# Autodesk Inventor assembly: Tiger
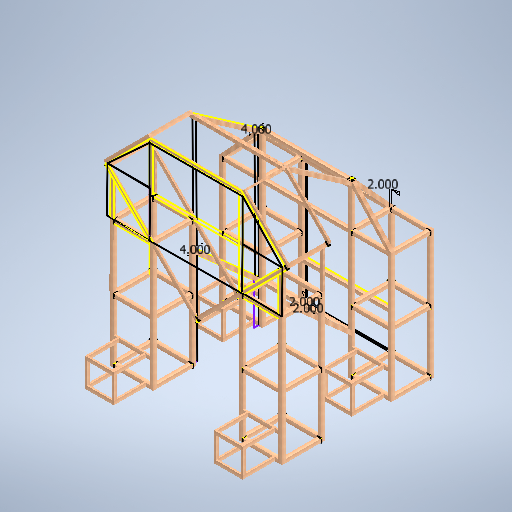
[picture p0: Inventor's stored thumbnail of the model, 512x512]
Saved by Autodesk Inventor 2025 (Build 290162000, 162)
## iProperties
Created: 2024-06-05
Part Number: Tiger
Document SubType Name: Assembly
Designer: Cupri
Mass: 180546 g
Surface Area: 136258 cm^2
Volume: 328266 cm^3
Density: 0.55 g/cm^3
Author: Cupri
## Documents named in this file (25)
- C:\Users\Cupri\OneDrive - University of South Carolina\Documents\Tiger\USCTigerBurn24\v2\Tiger.iam
- C:\Users\Cupri\OneDrive - University of South Carolina\Documents\Tiger\USCTigerBurn24\Standard Timber\4x4x72.ipt
- C:\Users\Cupri\OneDrive - University of South Carolina\Documents\Tiger\USCTigerBurn24\Standard Timber\4x4x40.ipt
- C:\Users\Cupri\OneDrive - University of South Carolina\Documents\Tiger\USCTigerBurn24\Standard Timber\2x4x36.ipt
- C:\Users\Cupri\OneDrive - University of South Carolina\Documents\Tiger\USCTigerBurn24\Standard Timber\2x4x40.ipt
- C:\Users\Cupri\OneDrive - University of South Carolina\Documents\Tiger\USCTigerBurn24\Standard Timber\2x4x24.ipt
- C:\Users\Cupri\OneDrive - University of South Carolina\Documents\Tiger\USCTigerBurn24\Standard Timber\2x4x28.ipt
- C:\Users\Cupri\OneDrive - University of South Carolina\Documents\Tiger\USCTigerBurn24\Standard Timber\2x4x72 (45 90).ipt
- C:\Users\Cupri\OneDrive - University of South Carolina\Documents\Tiger\USCTigerBurn24\Standard Timber\2x4x68 (45 90).ipt
- C:\Users\Cupri\OneDrive - University of South Carolina\Documents\Tiger\USCTigerBurn24\Standard Timber\2x4x42.343 (45 90).ipt
- C:\Users\Cupri\OneDrive - University of South Carolina\Documents\Tiger\USCTigerBurn24\Standard Timber\2x4x72 (30 90).ipt
- C:\Users\Cupri\OneDrive - University of South Carolina\Documents\Tiger\USCTigerBurn24\Standard Timber\2x4x44.ipt
- C:\Users\Cupri\OneDrive - University of South Carolina\Documents\Tiger\USCTigerBurn24\Standard Timber\4x4x104.303.ipt
- C:\Users\Cupri\OneDrive - University of South Carolina\Documents\Tiger\USCTigerBurn24\Standard Timber\4x4xidkanymore.ipt
- C:\Users\Cupri\OneDrive - University of South Carolina\Documents\Tiger\USCTigerBurn24\Standard Timber\4x4x48.ipt
- C:\Users\Cupri\OneDrive - University of South Carolina\Documents\Tiger\USCTigerBurn24\Standard Timber\4x4xigiveup.ipt
- C:\Users\Cupri\OneDrive - University of South Carolina\Documents\Tiger\USCTigerBurn24\Standard Timber\4x4x96.ipt
- C:\Users\Cupri\OneDrive - University of South Carolina\Documents\Tiger\USCTigerBurn24\Standard Timber\2x4x96.ipt
- C:\Users\Cupri\OneDrive - University of South Carolina\Documents\Tiger\USCTigerBurn24\Standard Timber\2x4xidk.ipt
- C:\Users\Cupri\OneDrive - University of South Carolina\Documents\Tiger\USCTigerBurn24\v2\Tiger\AIP\FEA\epzzwi8io.fins
- C:\Users\Cupri\OneDrive - University of South Carolina\Documents\Tiger\USCTigerBurn24\v2\Tiger\AIP\FEA\epzzwi8io.fsat
- C:\Users\Cupri\OneDrive - University of South Carolina\Documents\Tiger\USCTigerBurn24\v2\Tiger\AIP\FEA\epzzwi8io.ftes
- C:\Users\Cupri\OneDrive - University of South Carolina\Documents\Tiger\USCTigerBurn24\v2\Tiger\AIP\FEA\epzzwi8io.fwiz
- C:\Users\Cupri\OneDrive - University of South Carolina\Documents\Tiger\USCTigerBurn24\v2\Tiger\AIP\FEA\epzzwi8jk.fmsh
- C:\Users\Cupri\OneDrive - University of South Carolina\Documents\Tiger\USCTigerBurn24\v2\Tiger\AIP\FEA\epzzwi8jl.fres
## Components (160 placed, 18 different names)
1. 4x4x72:33 — Flush:163, Mate:149, Flush:164, Mate:182, Flush:229
2. 4x4x72:34 — Flush:161, Mate:148, Flush:162
3. 4x4x40:65
4. 4x4x40:66
5. 4x4x40:67
6. 4x4x40:68 — Flush:168
7. 4x4x40:69 — Flush:161
8. 4x4x40:70
9. 4x4x40:71
10. 4x4x40:72
11. 4x4x72:35 — Mate:150, Flush:165, Flush:166, Flush:224, Mate:181, Flush:227, Flush:228
12. 4x4x72:36 — Flush:158
13. 2x4x40:3
14. 2x4x36:9 — Mate:151
15. 2x4x36:10 — Flush:169, Flush:170
16. 2x4x36:11
17. 2x4x36:12
18. 2x4x24:5 — Flush:169
19. 2x4x24:6
20. 2x4x28:5 — Flush:170, Flush:200
21. 2x4x28:6 — Flush:167, Mate:151
22. 4x4x72:37 — Flush:163, Mate:149, Flush:164, Rigid:148, Flush:210, Mate:183, Flush:234
23. 4x4x72:38 — Mate:148, Flush:162
24. 4x4x40:77
25. 4x4x40:78
26. 4x4x40:79
27. 4x4x40:80 — Flush:231
28. 4x4x72:39 — Mate:150, Flush:165, Flush:166, Mate:172, Flush:215, Flush:216, Mate:184
29. 4x4x72:40 — Flush:158, Mate:173
30. 4x4x72:41
31. 4x4x72:42
32. 4x4x40:81
33. 4x4x40:82 — Flush:198
34. 4x4x40:83 — Flush:199
35. 4x4x40:84
36. 4x4x40:85
37. 4x4x40:86
38. 4x4x40:87
39. 4x4x40:88
40. 4x4x72:43
41. 4x4x72:44 — Flush:223
42. 2x4x40:4
43. 2x4x36:13
44. 2x4x36:14
45. 2x4x36:15
46. 2x4x36:16
47. 2x4x24:7
48. 2x4x24:8
49. 2x4x28:7 — Flush:200
50. 2x4x28:8
51. 4x4x72:45 — Flush:207
52. 4x4x72:46 — Flush:205, Rigid:147, Flush:211
53. 4x4x40:89 — Flush:206, Flush:212
54. 4x4x40:90 — Flush:208, Flush:209, Mate:176
55. 4x4x40:91 — Flush:205, Flush:207
56. 4x4x40:92 — Flush:206
57. 4x4x72:47 — Flush:208
58. 4x4x72:48 — Flush:209, Mate:171, Flush:213, Flush:214
59. 4x4x104.303:1 — Flush:221, Flush:222, Flush:224
60. 4x4x104.303:2 — Mate:179, Flush:220, Flush:221, Flush:222, Flush:223
61. 4x4xidkanymore:1 — Rigid:147, Flush:211, Flush:212
62. 4x4xidkanymore:2 — Rigid:148, Flush:210
63. 4x4x48:1 — Mate:172, Flush:215, Flush:216, Mate:174, Flush:217, Mate:180, Flush:225, Rigid:149, Flush:233, Mate:185, Flush:235, Flush:236
64. 4x4x48:2 — Mate:171, Flush:213, Flush:214, Mate:175, Flush:218, Rigid:150, Flush:226
65. 4x4xidkanymore:3 — Mate:173, Mate:174, Flush:217
66. 4x4xidkanymore:4 — Mate:175, Flush:218, Mate:176
67. 4x4xigiveup:1 — Mate:180, Flush:225, Rigid:149, Mate:186
68. 4x4xigiveup:2 — Rigid:150, Flush:226, Flush:237, Mate:187, Mate:188
69. 4x4x96:1 — Mate:183, Flush:231, Flush:232, Flush:234
70. 4x4x96:2 — Mate:184, Flush:232, Flush:233
71. 4x4x96:3 — Mate:181, Flush:227, Flush:228, Flush:230
72. 4x4x96:4 — Mate:182, Flush:229, Flush:230
73. 4x4x96:5 — Mate:185, Flush:235, Flush:236
74. 2x4x96:1 — Mate:186, Flush:237, Mate:187, Mate:188, Mate:191
75. 2x4xidk:1 — Mate:189, Mate:190, Mate:191, Flush:241
76. 2x4xidk:2 — Mate:192, Flush:240, Flush:241
77. 4x4x72:1 — Rigid:1, Rigid:3, Rigid:10, Rigid:11, Flush:39
78. 4x4x72:2 — Rigid:2, Rigid:4, Rigid:8
79. 4x4x40:1 — Rigid:1, Rigid:2
80. 4x4x40:2 — Rigid:3, Rigid:5, Flush:38, Mate:36
81. 4x4x40:3 — Rigid:6, Mate:5, Mate:6, Flush:4, Flush:5, Flush:19, Flush:20
82. 4x4x40:4 — Rigid:4, Rigid:7
83. 4x4x40:5 — Rigid:8
84. 4x4x40:6 — Rigid:9
85. 4x4x40:7 — Rigid:11
86. 4x4x40:8 — Rigid:10
87. 4x4x72:3 — Rigid:5, Rigid:6, Rigid:9, Mate:4, Flush:3, Mate:81
88. 4x4x72:4 — Rigid:7, Mate:7, Flush:21, Flush:22, Flush:159, Flush:160
89. 4x4x40:9
90. 4x4x40:10
91. 4x4x40:12 — Flush:168
92. 2x4x40:1 — Mate:4, Flush:3, Mate:5, Mate:8, Flush:6, Mate:9, Flush:7, Flush:17, Flush:18, Mate:81
93. 2x4x36:1 — Mate:6, Flush:4, Rigid:24, Flush:19, Flush:23
94. 2x4x36:2 — Mate:8, Flush:6, Flush:17, Mate:26, Mate:82
95. 2x4x36:3 — Mate:9, Flush:7, Mate:10, Rigid:26, Flush:18, Flush:21
96. 2x4x36:4 — Mate:7, Flush:5, Mate:10, Rigid:25, Rigid:27, Flush:20, Flush:22
97. 2x4x24:1 — Rigid:24, Mate:82
98. 2x4x24:2 — Rigid:25
99. 2x4x28:1 — Rigid:26, Mate:26
100. 2x4x28:2 — Rigid:27, Flush:23, Flush:167
101. 4x4x72:17 — Mate:62, Flush:65, Mate:63, Flush:91, Flush:92
102. 4x4x72:18 — Mate:64, Flush:66, Flush:90, Mate:76
103. 4x4x40:37 — Mate:75, Flush:89, Flush:90, Mate:76
104. 4x4x40:38 — Flush:85, Flush:86, Mate:74
105. 4x4x40:39 — Flush:92
106. 4x4x40:40 — Flush:91
107. 4x4x72:19 — Mate:38, Flush:41, Rigid:105, Mate:41, Flush:43, Flush:45, Flush:83, Flush:84, Flush:85
108. 4x4x72:20 — Mate:44, Flush:49, Flush:86, Flush:87, Mate:74, Mate:75, Flush:89, Flush:159, Flush:160
109. 4x4x72:21
110. 4x4x72:22 — Flush:39, Mate:77, Mate:179
111. 4x4x40:41
112. 4x4x40:42 — Flush:198
113. 4x4x40:43
114. 4x4x40:44 — Flush:38, Mate:36
115. 4x4x40:45
116. 4x4x40:46
117. 4x4x40:47
118. 4x4x40:48
119. 4x4x72:23 — Mate:78
120. 4x4x72:24
121. 4x4x40:49 — Flush:199
122. 4x4x40:50
123. 4x4x40:52
124. 2x4x40:2 — Mate:78, Mate:79, Mate:80
125. 2x4x36:5
126. 2x4x36:6 — Flush:50, Mate:47, Mate:80, Flush:95, Flush:96
127. 2x4x36:7 — Flush:93, Flush:94
128. 2x4x36:8
129. 2x4x24:3 — Mate:79
130. 2x4x24:4 — Flush:93, Flush:94
131. 2x4x28:3 — Flush:50, Mate:47, Flush:95, Flush:96
132. 2x4x28:4
133. 4x4x72:29 — Mate:57, Flush:57, Flush:58
134. 4x4x72:30 — Mate:58, Mate:60, Flush:60, Mate:77, Mate:178, Flush:220
135. 4x4x40:61
136. 4x4x40:62 — Flush:79, Flush:81, Mate:72
137. 4x4x40:63 — Flush:219, Mate:177, Mate:178
138. 4x4x40:64 — Mate:73
139. 4x4x72:31 — Mate:42, Mate:43, Flush:46, Flush:47, Flush:78, Flush:79, Mate:72, Mate:73
140. 4x4x72:32 — Mate:37, Flush:40, Rigid:104, Mate:39, Mate:40, Flush:42, Flush:80, Flush:81, Flush:82
141. 2x4x72 (45 90):1 — Mate:37, Flush:40, Rigid:104, Flush:80, Flush:88
142. 2x4x68 (45 90):1 — Mate:38, Flush:41, Rigid:105, Flush:44, Flush:83, Flush:88
143. 2x4x72 (45 90):2 — Mate:39, Mate:40, Flush:42, Flush:48, Mate:48, Flush:51, Mate:49, Flush:82
144. 2x4x72 (45 90):3 — Mate:41, Flush:43, Flush:44, Flush:45, Mate:45, Mate:50, Flush:52, Mate:51, Flush:84
145. 2x4x42.343 (45 90):1 — Mate:42, Mate:43, Flush:46, Flush:47, Flush:48, Flush:78
146. 2x4x42.343 (45 90):2 — Mate:44, Mate:45, Flush:49, Flush:87
147. 2x4x72 (30 90):1 — Mate:48, Flush:51, Mate:49, Flush:70, Flush:238, Mate:192, Flush:240
148. 2x4x72 (30 90):2 — Mate:50, Flush:52, Mate:51, Flush:71, Flush:72
149. 2x4x72 (45 90):4 — Mate:60, Flush:60, Mate:61, Flush:61, Flush:62
150. 2x4x68 (45 90):2 — Mate:61, Flush:61, Flush:62
151. 2x4x72 (45 90):5 — Flush:59, Mate:58, Mate:59, Mate:65, Flush:67, Flush:68, Flush:219, Mate:177
152. 2x4x72 (45 90):6 — Flush:63, Flush:64, Mate:62, Flush:65, Mate:63, Mate:68, Flush:73
153. 2x4x42.343 (45 90):3 — Mate:57, Flush:57, Flush:58, Flush:59, Mate:59
154. 2x4x42.343 (45 90):4 — Flush:63, Mate:64, Flush:66
155. 2x4x72 (30 90):3 — Mate:66, Flush:69, Flush:204, Mate:189
156. 2x4x72 (30 90):4 — Flush:64, Mate:67, Mate:69, Flush:239
157. 2x4x44:1 — Mate:67, Flush:71, Flush:72, Flush:239, Mate:190
158. 2x4x44:2 — Mate:65, Flush:67, Flush:68
159. 2x4x44:3 — Mate:66, Flush:69, Flush:70, Flush:204, Flush:238
160. 2x4x44:4 — Mate:68, Flush:73, Mate:69
## Relationships (372: Flush 176, Mate 114, WeldJoint 82)
- Rigid:1 [WeldJoint]: 4x4x72:1 ↔ 4x4x40:1
- Rigid:2 [WeldJoint]: 4x4x72:2 ↔ 4x4x40:1
- Rigid:3 [WeldJoint]: 4x4x72:1 ↔ 4x4x40:2
- Rigid:4 [WeldJoint]: 4x4x72:2 ↔ 4x4x40:4
- Rigid:5 [WeldJoint]: 4x4x40:2 ↔ 4x4x72:3
- Rigid:6 [WeldJoint]: 4x4x40:3 ↔ 4x4x72:3
- Rigid:7 [WeldJoint]: 4x4x40:4 ↔ 4x4x72:4
- Rigid:8 [WeldJoint]: 4x4x72:2 ↔ 4x4x40:5
- Rigid:9 [WeldJoint]: 4x4x40:6 ↔ 4x4x72:3
- Rigid:10 [WeldJoint]: 4x4x72:1 ↔ 4x4x40:8
- Rigid:11 [WeldJoint]: 4x4x72:1 ↔ 4x4x40:7
- Mate:4: 4x4x72:3 ↔ 2x4x40:1
- Flush:3: 4x4x72:3 ↔ 2x4x40:1
- Mate:5 (609.6 mm): 4x4x40:3 ↔ 2x4x40:1
- Mate:6 (101.6 mm): 4x4x40:3 ↔ 2x4x36:1
- Flush:4: 4x4x40:3 ↔ 2x4x36:1
- Mate:7 (101.6 mm): 4x4x72:4 ↔ 2x4x36:4
- Flush:5: 4x4x40:3 ↔ 2x4x36:4
- Mate:8 (101.6 mm): 2x4x40:1 ↔ 2x4x36:2
- Flush:6: 2x4x40:1 ↔ 2x4x36:2
- Mate:9: 2x4x40:1 ↔ 2x4x36:3
- Flush:7: 2x4x40:1 ↔ 2x4x36:3
- Mate:10: 2x4x36:3 ↔ 2x4x36:4
- Rigid:24 [WeldJoint]: 2x4x36:1 ↔ 2x4x24:1
- Rigid:25 [WeldJoint]: 2x4x36:4 ↔ 2x4x24:2
- Rigid:26 [WeldJoint]: 2x4x36:3 ↔ 2x4x28:1
- Rigid:27 [WeldJoint]: 2x4x36:4 ↔ 2x4x28:2
- [WeldJoint]: 4x4x72:18 ↔ 4x4x40:37
- [WeldJoint]: 4x4x40:38 ↔ 4x4x72:19
- [WeldJoint]: 4x4x72:17 ↔ 4x4x40:40
- [WeldJoint]: 4x4x72:17 ↔ 4x4x40:39
- Flush:17: 2x4x40:1 ↔ 2x4x36:2
- Flush:18: 2x4x40:1 ↔ 2x4x36:3
- Flush:19: 4x4x40:3 ↔ 2x4x36:1
- Flush:20: 4x4x40:3 ↔ 2x4x36:4
- Flush:21 (203.2 mm): 4x4x72:4 ↔ 2x4x36:3
- Flush:22 (203.2 mm): 4x4x72:4 ↔ 2x4x36:4
- Flush:23: 2x4x36:1 ↔ 2x4x28:2
- Mate:26: 2x4x36:2 ↔ 2x4x28:1
- [WeldJoint]: 4x4x72:21 ↔ 4x4x40:41
- [WeldJoint]: 4x4x72:22 ↔ 4x4x40:41
- [WeldJoint]: 4x4x72:21 ↔ 4x4x40:42
- [WeldJoint]: 4x4x72:22 ↔ 4x4x40:44
- [WeldJoint]: 4x4x40:42 ↔ 4x4x72:23
- [WeldJoint]: 4x4x40:43 ↔ 4x4x72:23
- [WeldJoint]: 4x4x40:44 ↔ 4x4x72:24
- [WeldJoint]: 4x4x72:22 ↔ 4x4x40:45
- [WeldJoint]: 4x4x40:46 ↔ 4x4x72:23
- [WeldJoint]: 4x4x72:21 ↔ 4x4x40:48
- [WeldJoint]: 4x4x72:21 ↔ 4x4x40:47
- [Mate]: 4x4x72:23 ↔ 2x4x40:2
- [Flush]: 4x4x72:23 ↔ 2x4x40:2
- [Mate] (609.6 mm): 4x4x40:43 ↔ 2x4x40:2
- [Mate] (101.6 mm): 4x4x40:43 ↔ 2x4x36:5
- [Flush]: 4x4x40:43 ↔ 2x4x36:5
- [Mate] (101.6 mm): 4x4x72:24 ↔ 2x4x36:8
- [Flush]: 4x4x40:43 ↔ 2x4x36:8
- [Mate]: 2x4x40:2 ↔ 2x4x36:7
- [Flush]: 2x4x40:2 ↔ 2x4x36:7
- [Mate]: 2x4x36:7 ↔ 2x4x36:8
- [WeldJoint]: 2x4x36:5 ↔ 2x4x24:3
- [WeldJoint]: 2x4x36:8 ↔ 2x4x24:4
- [WeldJoint]: 2x4x36:7 ↔ 2x4x28:3
- [WeldJoint]: 2x4x36:8 ↔ 2x4x28:4
- [WeldJoint]: 4x4x72:30 ↔ 4x4x40:61
- [WeldJoint]: 4x4x40:62 ↔ 4x4x72:31
- [WeldJoint]: 4x4x72:29 ↔ 4x4x40:64
- [WeldJoint]: 4x4x72:29 ↔ 4x4x40:63
- [Flush]: 2x4x40:2 ↔ 2x4x36:7
- [Flush]: 4x4x40:43 ↔ 2x4x36:5
- [Flush]: 4x4x40:43 ↔ 2x4x36:8
- [Flush] (203.2 mm): 4x4x72:24 ↔ 2x4x36:7
- [Flush] (203.2 mm): 4x4x72:24 ↔ 2x4x36:8
- [Flush]: 2x4x36:5 ↔ 2x4x28:4
- Flush:38: 4x4x40:2 ↔ 4x4x40:44
- Flush:39: 4x4x72:1 ↔ 4x4x72:22
- Mate:36 (2438.4 mm): 4x4x40:2 ↔ 4x4x40:44
- Mate:37: 4x4x72:32 ↔ 2x4x72 (45 90):1
- Flush:40: 4x4x72:32 ↔ 2x4x72 (45 90):1
- Rigid:104 [WeldJoint]: 4x4x72:32 ↔ 2x4x72 (45 90):1
- Mate:38: 4x4x72:19 ↔ 2x4x68 (45 90):1
- Flush:41: 4x4x72:19 ↔ 2x4x68 (45 90):1
- Rigid:105 [WeldJoint]: 4x4x72:19 ↔ 2x4x68 (45 90):1
- Mate:39: 4x4x72:32 ↔ 2x4x72 (45 90):2
- Mate:40: 4x4x72:32 ↔ 2x4x72 (45 90):2
- Flush:42: 4x4x72:32 ↔ 2x4x72 (45 90):2
- Mate:41: 4x4x72:19 ↔ 2x4x72 (45 90):3
- Flush:43: 4x4x72:19 ↔ 2x4x72 (45 90):3
- Flush:44: 2x4x68 (45 90):1 ↔ 2x4x72 (45 90):3
- Flush:45: 4x4x72:19 ↔ 2x4x72 (45 90):3
- Mate:42: 4x4x72:31 ↔ 2x4x42.343 (45 90):1
- Mate:43: 4x4x72:31 ↔ 2x4x42.343 (45 90):1
- Flush:46: 4x4x72:31 ↔ 2x4x42.343 (45 90):1
- Flush:47: 4x4x72:31 ↔ 2x4x42.343 (45 90):1
- Flush:48: 2x4x72 (45 90):2 ↔ 2x4x42.343 (45 90):1
- Mate:44: 4x4x72:20 ↔ 2x4x42.343 (45 90):2
- Mate:45: 2x4x72 (45 90):3 ↔ 2x4x42.343 (45 90):2
- Flush:49: 4x4x72:20 ↔ 2x4x42.343 (45 90):2
- Flush:50: 2x4x36:6 ↔ 2x4x28:3
- Mate:47: 2x4x36:6 ↔ 2x4x28:3
- Mate:48: 2x4x72 (45 90):2 ↔ 2x4x72 (30 90):1
- Flush:51: 2x4x72 (45 90):2 ↔ 2x4x72 (30 90):1
- Mate:49: 2x4x72 (45 90):2 ↔ 2x4x72 (30 90):1
- Mate:50: 2x4x72 (45 90):3 ↔ 2x4x72 (30 90):2
- Flush:52: 2x4x72 (45 90):3 ↔ 2x4x72 (30 90):2
- Mate:51: 2x4x72 (45 90):3 ↔ 2x4x72 (30 90):2
- [Flush]: 2x4x68 (45 90):2 ↔ 2x4x72 (45 90):6
- [Flush]: 2x4x72 (45 90):5 ↔ 2x4x42.343 (45 90):3
- [Mate]: 2x4x72 (45 90):6 ↔ 2x4x42.343 (45 90):4
- [Mate]: 2x4x72 (45 90):5 ↔ 2x4x72 (30 90):3
- [Flush]: 2x4x72 (45 90):5 ↔ 2x4x72 (30 90):3
- [Mate]: 2x4x72 (45 90):5 ↔ 2x4x72 (30 90):3
- [Mate]: 2x4x72 (45 90):6 ↔ 2x4x72 (30 90):4
- [Flush]: 2x4x72 (45 90):6 ↔ 2x4x72 (30 90):4
- [Mate]: 2x4x72 (45 90):6 ↔ 2x4x72 (30 90):4
- Mate:57: 4x4x72:29 ↔ 2x4x42.343 (45 90):3
- Flush:57: 4x4x72:29 ↔ 2x4x42.343 (45 90):3
- Flush:58: 4x4x72:29 ↔ 2x4x42.343 (45 90):3
- Flush:59: 2x4x72 (45 90):5 ↔ 2x4x42.343 (45 90):3
- Mate:58: 4x4x72:30 ↔ 2x4x72 (45 90):5
- Mate:59: 2x4x72 (45 90):5 ↔ 2x4x42.343 (45 90):3
- Mate:60: 4x4x72:30 ↔ 2x4x72 (45 90):4
- Flush:60: 4x4x72:30 ↔ 2x4x72 (45 90):4
- Mate:61: 2x4x72 (45 90):4 ↔ 2x4x68 (45 90):2
- Flush:61: 2x4x72 (45 90):4 ↔ 2x4x68 (45 90):2
- Flush:62: 2x4x72 (45 90):4 ↔ 2x4x68 (45 90):2
- Flush:63: 2x4x72 (45 90):6 ↔ 2x4x42.343 (45 90):4
- Flush:64: 2x4x72 (45 90):6 ↔ 2x4x72 (30 90):4
- Mate:62: 4x4x72:17 ↔ 2x4x72 (45 90):6
- Flush:65: 4x4x72:17 ↔ 2x4x72 (45 90):6
- Mate:63: 4x4x72:17 ↔ 2x4x72 (45 90):6
- Mate:64: 4x4x72:18 ↔ 2x4x42.343 (45 90):4
- Flush:66: 4x4x72:18 ↔ 2x4x42.343 (45 90):4
- Mate:65: 2x4x72 (45 90):5 ↔ 2x4x44:2
- Flush:67: 2x4x72 (45 90):5 ↔ 2x4x44:2
- Flush:68: 2x4x72 (45 90):5 ↔ 2x4x44:2
- Mate:66: 2x4x72 (30 90):3 ↔ 2x4x44:3
- Flush:69: 2x4x72 (30 90):3 ↔ 2x4x44:3
- Flush:70: 2x4x72 (30 90):1 ↔ 2x4x44:3
- Mate:67: 2x4x72 (30 90):4 ↔ 2x4x44:1
- Flush:71: 2x4x72 (30 90):2 ↔ 2x4x44:1
- Flush:72: 2x4x72 (30 90):2 ↔ 2x4x44:1
- Mate:68: 2x4x72 (45 90):6 ↔ 2x4x44:4
- Flush:73: 2x4x72 (45 90):6 ↔ 2x4x44:4
- Mate:69: 2x4x72 (30 90):4 ↔ 2x4x44:4
- Flush:78: 4x4x72:31 ↔ 2x4x42.343 (45 90):1
- Flush:79: 4x4x40:62 ↔ 4x4x72:31
- Flush:80: 4x4x72:32 ↔ 2x4x72 (45 90):1
- Flush:81: 4x4x40:62 ↔ 4x4x72:32
- Flush:82: 4x4x72:32 ↔ 2x4x72 (45 90):2
- Flush:83: 4x4x72:19 ↔ 2x4x68 (45 90):1
- Flush:84: 4x4x72:19 ↔ 2x4x72 (45 90):3
- Flush:85: 4x4x40:38 ↔ 4x4x72:19
- Flush:86: 4x4x40:38 ↔ 4x4x72:20
- Flush:87: 4x4x72:20 ↔ 2x4x42.343 (45 90):2
- Flush:88: 2x4x72 (45 90):1 ↔ 2x4x68 (45 90):1
- Mate:72: 4x4x40:62 ↔ 4x4x72:31
- Mate:73: 4x4x40:64 ↔ 4x4x72:31
- Mate:74: 4x4x40:38 ↔ 4x4x72:20
- Mate:75: 4x4x40:37 ↔ 4x4x72:20
- Flush:89: 4x4x40:37 ↔ 4x4x72:20
- Flush:90: 4x4x72:18 ↔ 4x4x40:37
- Mate:76: 4x4x72:18 ↔ 4x4x40:37
- Flush:91: 4x4x72:17 ↔ 4x4x40:40
- Flush:92: 4x4x72:17 ↔ 4x4x40:39
- Mate:77: 4x4x72:22 ↔ 4x4x72:30
- Mate:78: 4x4x72:23 ↔ 2x4x40:2
- Mate:79: 2x4x40:2 ↔ 2x4x24:3
- Flush:93: 2x4x36:7 ↔ 2x4x24:4
- Flush:94: 2x4x36:7 ↔ 2x4x24:4
- Mate:80: 2x4x40:2 ↔ 2x4x36:6
- Flush:95: 2x4x36:6 ↔ 2x4x28:3
- Flush:96: 2x4x36:6 ↔ 2x4x28:3
- Mate:81: 4x4x72:3 ↔ 2x4x40:1
- Mate:82: 2x4x36:2 ↔ 2x4x24:1
- [WeldJoint]: 4x4x72:33 ↔ 4x4x40:65
- [WeldJoint]: 4x4x72:34 ↔ 4x4x40:65
- [WeldJoint]: 4x4x72:33 ↔ 4x4x40:66
- [WeldJoint]: 4x4x72:34 ↔ 4x4x40:68
- [WeldJoint]: 4x4x40:66 ↔ 4x4x72:35
- [WeldJoint]: 4x4x40:67 ↔ 4x4x72:35
- [WeldJoint]: 4x4x40:68 ↔ 4x4x72:36
- [WeldJoint]: 4x4x72:34 ↔ 4x4x40:69
- [WeldJoint]: 4x4x40:70 ↔ 4x4x72:35
- [WeldJoint]: 4x4x72:33 ↔ 4x4x40:72
- [WeldJoint]: 4x4x72:33 ↔ 4x4x40:71
- [Mate]: 4x4x72:35 ↔ 2x4x40:3
- [Flush]: 4x4x72:35 ↔ 2x4x40:3
- [Mate] (609.6 mm): 4x4x40:67 ↔ 2x4x40:3
- [Mate] (101.6 mm): 4x4x40:67 ↔ 2x4x36:9
- [Flush]: 4x4x40:67 ↔ 2x4x36:9
- [Mate] (101.6 mm): 4x4x72:36 ↔ 2x4x36:12
- [Flush]: 4x4x40:67 ↔ 2x4x36:12
- [Mate] (101.6 mm): 2x4x40:3 ↔ 2x4x36:10
- [Flush]: 2x4x40:3 ↔ 2x4x36:10
- [Mate]: 2x4x40:3 ↔ 2x4x36:11
- [Flush]: 2x4x40:3 ↔ 2x4x36:11
- [Mate]: 2x4x36:11 ↔ 2x4x36:12
- [WeldJoint]: 2x4x36:9 ↔ 2x4x24:5
- [WeldJoint]: 2x4x36:12 ↔ 2x4x24:6
- [WeldJoint]: 2x4x36:11 ↔ 2x4x28:5
- [WeldJoint]: 2x4x36:12 ↔ 2x4x28:6
- [WeldJoint]: 4x4x72:38 ↔ 4x4x40:77
- [WeldJoint]: 4x4x40:78 ↔ 4x4x72:39
- [WeldJoint]: 4x4x72:37 ↔ 4x4x40:80
- [WeldJoint]: 4x4x72:37 ↔ 4x4x40:79
- [Flush]: 2x4x40:3 ↔ 2x4x36:10
- [Flush]: 2x4x40:3 ↔ 2x4x36:11
- [Flush]: 4x4x40:67 ↔ 2x4x36:9
- [Flush]: 4x4x40:67 ↔ 2x4x36:12
- [Flush] (203.2 mm): 4x4x72:36 ↔ 2x4x36:11
- [Flush] (203.2 mm): 4x4x72:36 ↔ 2x4x36:12
- [Flush]: 2x4x36:9 ↔ 2x4x28:6
- [Mate]: 2x4x36:10 ↔ 2x4x28:5
- [Flush]: 4x4x40:78 ↔ 4x4x72:39
- [Flush]: 4x4x40:78 ↔ 4x4x72:40
- [Mate]: 4x4x40:78 ↔ 4x4x72:40
- [Mate]: 4x4x40:77 ↔ 4x4x72:40
- [Flush]: 4x4x40:77 ↔ 4x4x72:40
- [Flush]: 4x4x72:38 ↔ 4x4x40:77
- [Mate]: 4x4x72:38 ↔ 4x4x40:77
- [Flush]: 4x4x72:37 ↔ 4x4x40:80
- [Flush]: 4x4x72:37 ↔ 4x4x40:79
- [Mate]: 4x4x72:35 ↔ 2x4x40:3
- [Mate]: 2x4x36:10 ↔ 2x4x24:5
- Flush:158: 4x4x72:36 ↔ 4x4x72:40
- Flush:159: 4x4x72:4 ↔ 4x4x72:20
- Flush:160: 4x4x72:4 ↔ 4x4x72:20
- Flush:161: 4x4x72:34 ↔ 4x4x40:69
- Mate:148: 4x4x72:34 ↔ 4x4x72:38
- Flush:162: 4x4x72:34 ↔ 4x4x72:38
- Flush:163: 4x4x72:33 ↔ 4x4x72:37
- Mate:149: 4x4x72:33 ↔ 4x4x72:37
- Flush:164: 4x4x72:33 ↔ 4x4x72:37
- Mate:150: 4x4x72:35 ↔ 4x4x72:39
- Flush:165: 4x4x72:35 ↔ 4x4x72:39
- Flush:166: 4x4x72:35 ↔ 4x4x72:39
- Flush:167: 2x4x28:6 ↔ 2x4x28:2
- Flush:168: 4x4x40:68 ↔ 4x4x40:12
- Mate:151: 2x4x36:9 ↔ 2x4x28:6
- Flush:169: 2x4x36:10 ↔ 2x4x24:5
- Flush:170: 2x4x36:10 ↔ 2x4x28:5
- [WeldJoint]: 4x4x72:41 ↔ 4x4x40:81
- [WeldJoint]: 4x4x72:42 ↔ 4x4x40:81
- [WeldJoint]: 4x4x72:41 ↔ 4x4x40:82
- [WeldJoint]: 4x4x72:42 ↔ 4x4x40:84
- [WeldJoint]: 4x4x40:82 ↔ 4x4x72:43
- [WeldJoint]: 4x4x40:83 ↔ 4x4x72:43
- [WeldJoint]: 4x4x40:84 ↔ 4x4x72:44
- [WeldJoint]: 4x4x72:42 ↔ 4x4x40:85
- [WeldJoint]: 4x4x40:86 ↔ 4x4x72:43
- [WeldJoint]: 4x4x72:41 ↔ 4x4x40:88
- [WeldJoint]: 4x4x72:41 ↔ 4x4x40:87
- [Mate]: 4x4x72:43 ↔ 2x4x40:4
- [Flush]: 4x4x72:43 ↔ 2x4x40:4
- [Mate] (609.6 mm): 4x4x40:83 ↔ 2x4x40:4
- [Mate] (101.6 mm): 4x4x40:83 ↔ 2x4x36:13
- [Flush]: 4x4x40:83 ↔ 2x4x36:13
- [Mate] (101.6 mm): 4x4x72:44 ↔ 2x4x36:16
- [Flush]: 4x4x40:83 ↔ 2x4x36:16
- [Mate] (101.6 mm): 2x4x40:4 ↔ 2x4x36:14
- [Flush]: 2x4x40:4 ↔ 2x4x36:14
- [Mate]: 2x4x40:4 ↔ 2x4x36:15
- [Flush]: 2x4x40:4 ↔ 2x4x36:15
- [Mate]: 2x4x36:15 ↔ 2x4x36:16
- [WeldJoint]: 2x4x36:13 ↔ 2x4x24:7
- [WeldJoint]: 2x4x36:16 ↔ 2x4x24:8
- [WeldJoint]: 2x4x36:15 ↔ 2x4x28:7
- [WeldJoint]: 2x4x36:16 ↔ 2x4x28:8
- [WeldJoint]: 4x4x72:46 ↔ 4x4x40:89
- [WeldJoint]: 4x4x40:90 ↔ 4x4x72:47
- [WeldJoint]: 4x4x72:45 ↔ 4x4x40:92
- [WeldJoint]: 4x4x72:45 ↔ 4x4x40:91
- [Flush]: 2x4x40:4 ↔ 2x4x36:14
- [Flush]: 2x4x40:4 ↔ 2x4x36:15
- [Flush]: 4x4x40:83 ↔ 2x4x36:13
- [Flush]: 4x4x40:83 ↔ 2x4x36:16
- [Flush] (203.2 mm): 4x4x72:44 ↔ 2x4x36:15
- [Flush] (203.2 mm): 4x4x72:44 ↔ 2x4x36:16
- [Flush]: 2x4x36:13 ↔ 2x4x28:8
- [Mate]: 2x4x36:14 ↔ 2x4x28:7
- [Flush]: 4x4x40:90 ↔ 4x4x72:47
- [Flush]: 4x4x40:90 ↔ 4x4x72:48
- [Mate]: 4x4x40:90 ↔ 4x4x72:48
- [Mate]: 4x4x40:89 ↔ 4x4x72:48
- [Flush]: 4x4x40:89 ↔ 4x4x72:48
- [Flush]: 4x4x72:46 ↔ 4x4x40:89
- [Mate]: 4x4x72:46 ↔ 4x4x40:89
- [Flush]: 4x4x72:45 ↔ 4x4x40:92
- [Flush]: 4x4x72:45 ↔ 4x4x40:91
- [Mate]: 4x4x72:43 ↔ 2x4x40:4
- [Mate]: 2x4x36:14 ↔ 2x4x24:7
- [Flush]: 4x4x72:44 ↔ 4x4x72:48
- [Flush]: 4x4x72:42 ↔ 4x4x40:85
- [Mate]: 4x4x72:42 ↔ 4x4x72:46
- [Flush]: 4x4x72:42 ↔ 4x4x72:46
- [Flush]: 4x4x72:41 ↔ 4x4x72:45
- [Mate]: 4x4x72:41 ↔ 4x4x72:45
- [Flush]: 4x4x72:41 ↔ 4x4x72:45
- [Mate]: 4x4x72:43 ↔ 4x4x72:47
- [Flush]: 4x4x72:43 ↔ 4x4x72:47
- [Flush]: 4x4x72:43 ↔ 4x4x72:47
- [Mate]: 2x4x36:13 ↔ 2x4x28:8
- [Flush]: 2x4x36:14 ↔ 2x4x24:7
- [Flush]: 2x4x36:14 ↔ 2x4x28:7
- Flush:198: 4x4x40:82 ↔ 4x4x40:42
- Flush:199: 4x4x40:83 ↔ 4x4x40:49
- Flush:200: 2x4x28:5 ↔ 2x4x28:7
- Flush:204: 2x4x72 (30 90):3 ↔ 2x4x44:3
- Flush:205: 4x4x72:46 ↔ 4x4x40:91
- Flush:206: 4x4x40:89 ↔ 4x4x40:92
- Flush:207: 4x4x72:45 ↔ 4x4x40:91
- Flush:208: 4x4x40:90 ↔ 4x4x72:47
- Flush:209: 4x4x40:90 ↔ 4x4x72:48
- Rigid:147 [WeldJoint]: 4x4x72:46 ↔ 4x4xidkanymore:1
- Rigid:148 [WeldJoint]: 4x4x72:37 ↔ 4x4xidkanymore:2
- Flush:210: 4x4x72:37 ↔ 4x4xidkanymore:2
- Flush:211: 4x4x72:46 ↔ 4x4xidkanymore:1
- Flush:212: 4x4x40:89 ↔ 4x4xidkanymore:1
- Mate:171: 4x4x72:48 ↔ 4x4x48:2
- Flush:213: 4x4x72:48 ↔ 4x4x48:2
- Flush:214: 4x4x72:48 ↔ 4x4x48:2
- Mate:172: 4x4x72:39 ↔ 4x4x48:1
- Flush:215: 4x4x72:39 ↔ 4x4x48:1
- Flush:216: 4x4x72:39 ↔ 4x4x48:1
- Mate:173: 4x4x72:40 ↔ 4x4xidkanymore:3
- Mate:174: 4x4x48:1 ↔ 4x4xidkanymore:3
- Flush:217: 4x4x48:1 ↔ 4x4xidkanymore:3
- Mate:175: 4x4x48:2 ↔ 4x4xidkanymore:4
- Flush:218: 4x4x48:2 ↔ 4x4xidkanymore:4
- Mate:176: 4x4x40:90 ↔ 4x4xidkanymore:4
- Flush:219: 4x4x40:63 ↔ 2x4x72 (45 90):5
- Mate:177: 4x4x40:63 ↔ 2x4x72 (45 90):5
- Mate:178: 4x4x72:30 ↔ 4x4x40:63
- Mate:179 (914.4 mm): 4x4x104.303:2 ↔ 4x4x72:22
- Flush:220: 4x4x104.303:2 ↔ 4x4x72:30
- Flush:221: 4x4x104.303:1 ↔ 4x4x104.303:2
- Flush:222: 4x4x104.303:1 ↔ 4x4x104.303:2
- Flush:223: 4x4x72:44 ↔ 4x4x104.303:2
- Flush:224: 4x4x72:35 ↔ 4x4x104.303:1
- Mate:180: 4x4x48:1 ↔ 4x4xigiveup:1
- Flush:225: 4x4x48:1 ↔ 4x4xigiveup:1
- Rigid:149 [WeldJoint]: 4x4x48:1 ↔ 4x4xigiveup:1
- Rigid:150 [WeldJoint]: 4x4x48:2 ↔ 4x4xigiveup:2
- Flush:226: 4x4x48:2 ↔ 4x4xigiveup:2
- Mate:181: 4x4x72:35 ↔ 4x4x96:3
- Flush:227: 4x4x72:35 ↔ 4x4x96:3
- Flush:228 (1053.8714 mm): 4x4x72:35 ↔ 4x4x96:3
- Mate:182: 4x4x72:33 ↔ 4x4x96:4
- Flush:229: 4x4x72:33 ↔ 4x4x96:4
- Flush:230: 4x4x96:3 ↔ 4x4x96:4
- Mate:183: 4x4x72:37 ↔ 4x4x96:1
- Mate:184: 4x4x72:39 ↔ 4x4x96:2
- Flush:231: 4x4x40:80 ↔ 4x4x96:1
- Flush:232: 4x4x96:1 ↔ 4x4x96:2
- Flush:233: 4x4x48:1 ↔ 4x4x96:2
- Flush:234: 4x4x72:37 ↔ 4x4x96:1
- Mate:185: 4x4x48:1 ↔ 4x4x96:5
- Flush:235: 4x4x48:1 ↔ 4x4x96:5
- Flush:236: 4x4x48:1 ↔ 4x4x96:5
- Mate:186: 4x4xigiveup:1 ↔ 2x4x96:1
- Flush:237: 4x4xigiveup:2 ↔ 2x4x96:1
- Mate:187: 4x4xigiveup:2 ↔ 2x4x96:1
- Mate:188: 4x4xigiveup:2 ↔ 2x4x96:1
- Flush:238: 2x4x72 (30 90):1 ↔ 2x4x44:3
- Flush:239: 2x4x72 (30 90):4 ↔ 2x4x44:1
- Mate:189: 2x4xidk:1 ↔ 2x4x72 (30 90):3
- Mate:190: 2x4xidk:1 ↔ 2x4x44:1
- Mate:191: 2x4x96:1 ↔ 2x4xidk:1
- Mate:192: 2x4xidk:2 ↔ 2x4x72 (30 90):1
- Flush:240: 2x4xidk:2 ↔ 2x4x72 (30 90):1
- Flush:241: 2x4xidk:1 ↔ 2x4xidk:2
## Named parameters: sa_0 = 22241.1, d136_d47_d36 = 0 mm, d137_d48_d37 = 0 mm, d138_d49_d38 = 0 mm, d139_d50_d39 = 0 mm, d154_d144 = 0 mm, d155_d145 = 0 mm, d156_d146 = 0 mm, d157_d147 = 203.2 mm, d158_d148 = 203.2 mm, d159_d149 = 0 mm, d168_d136_d47_d36 = 0 mm, d169_d137_d48_d37 = 0 mm, d170_d138_d49_d38 = 0 mm, d171_d139_d50_d39 = 0 mm, d173_d61 = 0 mm, d174_d62 = 0 mm, d175_d63 = 609.6 mm, d176_d68 = 101.6 mm, d177_d69 = 0 mm, d178_d70 = 101.6 mm, d179_d71 = 0 mm, d182_d74 = 0 mm, d183_d75 = 0 mm, d184_d76 = 0 mm, d185_d77 = 0 mm, d186_d78 = 0 mm, d187_d79 = 0 mm, d188_d80 = 0 mm, d190_d31 = 0 mm, d191_d32 = 0 mm, d192_d33 = 0 mm, d193_d34 = 0 mm, d194_d35 = 0 mm, d195_d36 = 0 mm, d196_d37 = 0 mm, d197_d38 = 0 mm, d198_d39 = 0 mm, d210_d29 = 0 mm, d211_d30 = 0 mm, d253_d234 = 0 mm, d254_d240 = 0 mm, d255_d242 = 0 mm, d256_d247 = 0 mm, d257_d248 = 0 mm, d258_d249 = 0 mm, d259_d250 = 0 mm, d260_d251 = 0 mm, d261_d252 = 0 mm, sa_1 = 980.999, d396_d137_d48_d37 = 0 mm, d397_d138_d49_d38 = 0 mm, d398_d139_d50_d39 = 0 mm, d399_d143 = 0 mm, d400_d144 = 0 mm, d401_d145 = 0 mm, d402_d146 = 0 mm, d403_d147 = 203.2 mm, d404_d148 = 203.2 mm, d405_d149 = 0 mm, d406_d150 = 0 mm, d407_d61 = 0 mm, d408_d62 = 0 mm, d409_d63 = 609.6 mm, d410_d68 = 101.6 mm, d411_d69 = 0 mm, d412_d70 = 101.6 mm, d413_d71 = 0 mm, d414_d72 = 101.6 mm, d415_d73 = 0 mm, d416_d74 = 0 mm, d417_d75 = 0 mm, d418_d76 = 0 mm, d419_d77 = 0 mm, d420_d78 = 0 mm, d421_d79 = 0 mm, d422_d80 = 0 mm, d423_d136_d47_d36 = 0 mm, d425_d31 = 0 mm, d426_d32 = 0 mm, d427_d33 = 0 mm, d428_d34 = 0 mm, d429_d35 = 0 mm, d430_d36 = 0 mm, d431_d37 = 0 mm, d432_d38 = 0 mm, d433_d39 = 0 mm, d434_d29 = 0 mm, d435_d30 = 0 mm, d436_d326 = 0 mm, d437_d327 = 0 mm, d438_d314 = 0 mm, d439_d315 = 0 mm, d440_d316 = 0 mm, d441_d317 = 0 mm, d442_d305 = 0 mm, d443_d306 = 0 mm, d444_d311 = 0 mm, d445_d312 = 0 mm, d446_d313 = 0 mm, d515_d433_d39 = 0 mm, d516_d434_d29 = 0 mm, d517_d435_d30 = 0 mm, d518_d436_d326 = 0 mm, d519_d437_d327 = 0 mm, d520_d438_d314 = 0 mm, d521_d439_d315 = 0 mm, d522_d440_d316 = 0 mm, d523_d441_d317 = 0 mm, d524_d442_d305 = 0 mm, d525_d443_d306 = 0 mm, d526_d444_d311 = 0 mm, d527_d445_d312 = 0 mm, d528_d446_d313 = 0 mm, d529_d396_d137_d48_d37 = 0 mm, d530_d397_d138_d49_d38 = 0 mm, d531_d398_d139_d50_d39 = 0 mm, d532_d399_d143 = 0 mm, d533_d400_d144 = 0 mm, d534_d401_d145 = 0 mm, d535_d402_d146 = 0 mm, d536_d403_d147 = 203.2 mm, d537_d404_d148 = 203.2 mm, d538_d405_d149 = 0 mm, d539_d406_d150 = 0 mm, d540_d407_d61 = 0 mm, d541_d408_d62 = 0 mm, d542_d409_d63 = 609.6 mm, d543_d410_d68 = 101.6 mm, d544_d411_d69 = 0 mm, d545_d412_d70 = 101.6 mm, d546_d413_d71 = 0 mm, d547_d414_d72 = 101.6 mm, d548_d415_d73 = 0 mm, d549_d416_d74 = 0 mm, d550_d417_d75 = 0 mm, d551_d418_d76 = 0 mm, d552_d419_d77 = 0 mm, d553_d420_d78 = 0 mm, d554_d421_d79 = 0 mm, d555_d422_d80 = 0 mm, d556_d423_d136_d47_d36 = 0 mm, d557_d425_d31 = 0 mm, d558_d426_d32 = 0 mm, d559_d427_d33 = 0 mm, d560_d428_d34 = 0 mm, d561_d429_d35 = 0 mm, d562_d430_d36 = 0 mm, d563_d431_d37 = 0 mm, d564_d432_d38 = 0 mm, d565_d505 = 0 mm, d566_d506 = 0 mm, d567_d507 = 0 mm, d568_d508 = 0 mm, d569_d509 = 0 mm, d570_d512 = 0 mm, d571_d513 = 0 mm, d572_d514 = 0 mm, d573_d498 = 0 mm, d574_d501 = 0 mm, d575_d502 = 0 mm, d576_d503 = 0 mm, d577_d504 = 0 mm
note: some values were not read from the file. Shown as the stored number, unit unknown: "sa_0", "sa_1".
